# Autodesk Inventor assembly: Printer Frame Assembly RevI
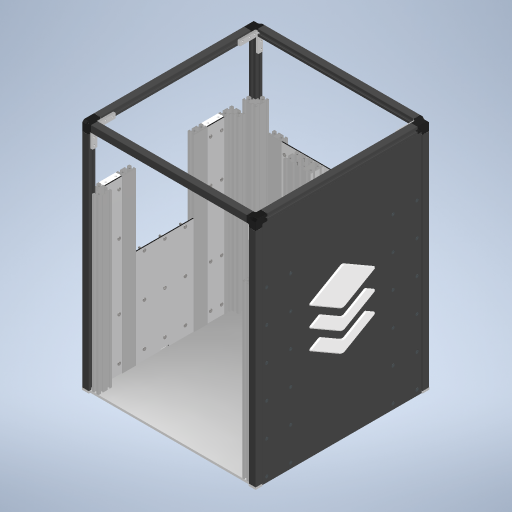
[picture p0: Inventor's stored thumbnail of the model, 512x512]
Saved by Autodesk Inventor 2024 (Build 280153000, 153)
## iProperties
Created: 2024-08-01
Part Number: Printer Frame Assembly RevI
Document SubType Name: Assembly
Designer: Ishaan
Author: Ishaan
## Documents named in this file (16)
- E:\Projects\Axiom--IDEX-3D-Printer\CAD\02 - Frame\Printer Frame Assembly RevI.iam
- E:\Projects\Axiom--IDEX-3D-Printer\CAD\02 - Frame\Printer Base Plate RevI.ipt
- E:\Projects\Axiom--IDEX-3D-Printer\CAD\00 - COTS Components\4040 Vertical L Extrusions\HFS5-404020-500.ipt
- E:\Projects\Axiom--IDEX-3D-Printer\CAD\00 - COTS Components\2040 Vertical Extrusions\HFSF5-2040-500.ipt
- E:\Projects\Axiom--IDEX-3D-Printer\CAD\00 - COTS Components\4080 Z-rail Extrusion\HFSP5-4080-500.ipt
- E:\Projects\Axiom--IDEX-3D-Printer\CAD\00 - COTS Components\2020 Frame Exterior Corners\HFSTB5-2020-650.ipt
- E:\Projects\Axiom--IDEX-3D-Printer\CAD\02 - Frame\Top Corner Extrusion Plate.ipt
- E:\Projects\Axiom--IDEX-3D-Printer\CAD\00 - COTS Components\2020 Frame Exterior X Runners\HFSTB5-2020-456.ipt
- E:\Projects\Axiom--IDEX-3D-Printer\CAD\00 - COTS Components\2020 Frame Exterior Y Runners\HFSFB5-2020-440.ipt
- E:\Projects\Axiom--IDEX-3D-Printer\CAD\02 - Frame\Exterior Frame Corner.ipt
- E:\Projects\Axiom--IDEX-3D-Printer\CAD\02 - Frame\Exterior Frame Corner Other.ipt
- E:\Projects\Axiom--IDEX-3D-Printer\CAD\08 - Side Panelling\Internal Narrow Panels.iam
- E:\Projects\Axiom--IDEX-3D-Printer\CAD\08 - Side Panelling\Internal Wide Panels.iam
- E:\Projects\Axiom--IDEX-3D-Printer\CAD\08 - Side Panelling\Internal Rear Panels.iam
- E:\Projects\Axiom--IDEX-3D-Printer\CAD\08 - Side Panelling\Exterior Side Panels.ipt
- E:\Projects\Axiom--IDEX-3D-Printer\CAD\00 - COTS Components\Hardware\FSCM5x8.ipt
## Components (62 placed, 15 different names)
1. Printer Base Plate RevI:1 — Insert:29, Flush:1, Insert:30, Flush:2, Insert:31, Flush:3, Insert:32, Flush:4, Insert:41, Insert:42, Insert:43, Insert:44, Insert:45, Insert:46, Insert:47, Insert:48, Insert:49, Insert:50, Insert:51, Insert:52, Insert:53, Insert:54, Insert:55, Insert:56, Insert:57, Insert:58, Mate:32
2. HFSF5-2040-500:1
3. HFSF5-2040-500:2 — Mate:33
4. HFSF5-2040-500:3 — Mate:30
5. HFSF5-2040-500:4 — Mate:31
6. HFS5-404020-500:1
7. HFS5-404020-500:2
8. HFS5-404020-500:3
9. HFS5-404020-500:4
10. HFS5-404020-500:5
11. HFS5-404020-500:6
12. HFSP5-4080-500:1 — Mate:29
13. HFSTB5-2020-650:1 — Mate:1, Flush:14, Insert:30, Flush:2, Mate:13
14. HFSTB5-2020-650:2 — Mate:3, Mate:11, Mate:12, Insert:29, Flush:1, Mate:34
15. HFSTB5-2020-650:3 — Mate:2, Flush:15, Insert:32, Flush:4, Mate:14
16. HFSTB5-2020-650:4 — Mate:4, Mate:5, Mate:6, Insert:31, Flush:3
17. Top Corner Extrusion Plate:1 — Mate:1, Flush:14, Mate:13, Insert:34, Angle:1, Mate:18, Insert:39, Mate:21
18. Top Corner Extrusion Plate:2 — Mate:2, Flush:15, Mate:14, Insert:35, Mate:16, Insert:40, Mate:22
19. Top Corner Extrusion Plate:3 — Mate:3, Mate:11, Mate:12, Insert:36, Angle:2, Mate:15, Insert:37, Mate:19
20. Top Corner Extrusion Plate:4 — Mate:4, Mate:5, Mate:6, Insert:33, Mate:17, Insert:38, Mate:20
21. HFSTB5-2020-456:1 — Insert:33, Insert:34, Angle:1
22. HFSTB5-2020-456:2 — Insert:35, Insert:36, Angle:2, Flush:16, Flush:17
23. HFSFB5-2020-440:1 — Mate:15, Flush:16, Mate:18, Mate:35
24. HFSFB5-2020-440:2 — Flush:17, Mate:16, Mate:17
25. Exterior Frame Corner:1 — Insert:37, Mate:19
26. Exterior Frame Corner:2 — Insert:38, Mate:20
27. Exterior Frame Corner Other:1 — Insert:39, Mate:21
28. Exterior Frame Corner Other:2 — Insert:40, Mate:22
29. HFSF5-2040-500:5 — Insert:43, Insert:44
30. HFSF5-2040-500:6 — Insert:41, Insert:42
31. Internal Narrow Panels:1 [sub-assembly] — Insert:51, Insert:52
32. Internal Narrow Panels:2 [sub-assembly] — Insert:49, Insert:50
33. Internal Narrow Panels:3 [sub-assembly] — Insert:47, Insert:48
34. Internal Narrow Panels:4 [sub-assembly] — Insert:45, Insert:46
35. Internal Wide Panels:1 [sub-assembly] — Insert:53, Insert:54, Insert:55
36. Internal Wide Panels:2 [sub-assembly] — Insert:56, Insert:57, Insert:58
37. Internal Rear Panels:1 [sub-assembly] — Mate:29, Mate:30, Mate:31, Mate:32
38. Exterior Side Panels:1 — Mate:33, Mate:34, Mate:35, Insert:59, Insert:60, Insert:61, Insert:62, Insert:63, Insert:64, Insert:65, Insert:66, Insert:67, Insert:68, Insert:69, Insert:70, Insert:71, Insert:72, Insert:73, Insert:74, Insert:75, Insert:76, Insert:77, Insert:78, Insert:79, Insert:80, Insert:81, Insert:82
39. FSCM5x8:1 — Insert:64
40. FSCM5x8:2 — Insert:63
41. FSCM5x8:3 — Insert:62
42. FSCM5x8:4 — Insert:61
43. FSCM5x8:5 — Insert:60
44. FSCM5x8:6 — Insert:59
45. FSCM5x8:7 — Insert:65
46. FSCM5x8:8 — Insert:66
47. FSCM5x8:9 — Insert:67
48. FSCM5x8:10 — Insert:68
49. FSCM5x8:11 — Insert:69
50. FSCM5x8:12 — Insert:70
51. FSCM5x8:13 — Insert:76
52. FSCM5x8:14 — Insert:75
53. FSCM5x8:15 — Insert:74
54. FSCM5x8:16 — Insert:73
55. FSCM5x8:17 — Insert:72
56. FSCM5x8:18 — Insert:71
57. FSCM5x8:19 — Insert:77
58. FSCM5x8:20 — Insert:78
59. FSCM5x8:21 — Insert:79
60. FSCM5x8:22 — Insert:80
61. FSCM5x8:23 — Insert:81
62. FSCM5x8:24 — Insert:82
## Relationships (117: Insert 82, Mate 25, Flush 8, Angle 2)
- [Insert]: Printer Base Plate RevI:1 ↔ HFSF5-2040-500:4
- [Insert]: Printer Base Plate RevI:1 ↔ HFSF5-2040-500:4
- [Insert]: Printer Base Plate RevI:1 ↔ HFSF5-2040-500:3
- [Insert]: Printer Base Plate RevI:1 ↔ HFSF5-2040-500:3
- [Insert]: Printer Base Plate RevI:1 ↔ HFSF5-2040-500:2
- [Insert]: Printer Base Plate RevI:1 ↔ HFSF5-2040-500:2
- [Insert]: Printer Base Plate RevI:1 ↔ HFSF5-2040-500:1
- [Insert]: Printer Base Plate RevI:1 ↔ HFSF5-2040-500:1
- [Insert]: Printer Base Plate RevI:1 ↔ HFS5-404020-500:6
- [Insert]: Printer Base Plate RevI:1 ↔ HFS5-404020-500:6
- [Insert]: Printer Base Plate RevI:1 ↔ HFS5-404020-500:5
- [Insert]: Printer Base Plate RevI:1 ↔ HFS5-404020-500:5
- [Insert]: Printer Base Plate RevI:1 ↔ HFS5-404020-500:4
- [Insert]: Printer Base Plate RevI:1 ↔ HFS5-404020-500:4
- [Insert]: Printer Base Plate RevI:1 ↔ HFS5-404020-500:3
- [Insert]: Printer Base Plate RevI:1 ↔ HFS5-404020-500:3
- [Insert]: Printer Base Plate RevI:1 ↔ HFS5-404020-500:2
- [Insert]: Printer Base Plate RevI:1 ↔ HFS5-404020-500:2
- [Insert]: Printer Base Plate RevI:1 ↔ HFS5-404020-500:1
- [Insert]: Printer Base Plate RevI:1 ↔ HFS5-404020-500:1
- [Insert]: Printer Base Plate RevI:1 ↔ HFSP5-4080-500:1
- [Insert]: Printer Base Plate RevI:1 ↔ HFSP5-4080-500:1
- [Insert]: Printer Base Plate RevI:1 ↔ HFSP5-4080-500:1
- [Insert]: Printer Base Plate RevI:1 ↔ HFSP5-4080-500:1
- [Insert]: Printer Base Plate RevI:1 ↔ HFSP5-4080-500:1
- [Insert]: Printer Base Plate RevI:1 ↔ HFSP5-4080-500:1
- [Insert]: Printer Base Plate RevI:1 ↔ HFSP5-4080-500:1
- [Insert]: Printer Base Plate RevI:1 ↔ HFSP5-4080-500:1
- Mate:1: HFSTB5-2020-650:1 ↔ Top Corner Extrusion Plate:1
- Mate:2: HFSTB5-2020-650:3 ↔ Top Corner Extrusion Plate:2
- Mate:3: HFSTB5-2020-650:2 ↔ Top Corner Extrusion Plate:3
- Mate:4: HFSTB5-2020-650:4 ↔ Top Corner Extrusion Plate:4
- Mate:5: HFSTB5-2020-650:4 ↔ Top Corner Extrusion Plate:4
- Mate:6 (9 mm): HFSTB5-2020-650:4 ↔ Top Corner Extrusion Plate:4
- Flush:14: HFSTB5-2020-650:1 ↔ Top Corner Extrusion Plate:1
- Flush:15: HFSTB5-2020-650:3 ↔ Top Corner Extrusion Plate:2
- Mate:11: HFSTB5-2020-650:2 ↔ Top Corner Extrusion Plate:3
- Mate:12 (9 mm): HFSTB5-2020-650:2 ↔ Top Corner Extrusion Plate:3
- Insert:29: Printer Base Plate RevI:1 ↔ HFSTB5-2020-650:2
- Flush:1: Printer Base Plate RevI:1 ↔ HFSTB5-2020-650:2
- Insert:30: Printer Base Plate RevI:1 ↔ HFSTB5-2020-650:1
- Flush:2: Printer Base Plate RevI:1 ↔ HFSTB5-2020-650:1
- Insert:31: Printer Base Plate RevI:1 ↔ HFSTB5-2020-650:4
- Flush:3: Printer Base Plate RevI:1 ↔ HFSTB5-2020-650:4
- Insert:32: Printer Base Plate RevI:1 ↔ HFSTB5-2020-650:3
- Flush:4: Printer Base Plate RevI:1 ↔ HFSTB5-2020-650:3
- Mate:13 (9 mm): HFSTB5-2020-650:1 ↔ Top Corner Extrusion Plate:1
- Mate:14 (9 mm): HFSTB5-2020-650:3 ↔ Top Corner Extrusion Plate:2
- Insert:33: Top Corner Extrusion Plate:4 ↔ HFSTB5-2020-456:1
- Insert:34: Top Corner Extrusion Plate:1 ↔ HFSTB5-2020-456:1
- Angle:1 (0 deg): Top Corner Extrusion Plate:1 ↔ HFSTB5-2020-456:1
- Insert:35: Top Corner Extrusion Plate:2 ↔ HFSTB5-2020-456:2
- Insert:36: Top Corner Extrusion Plate:3 ↔ HFSTB5-2020-456:2
- Angle:2 (0 deg): Top Corner Extrusion Plate:3 ↔ HFSTB5-2020-456:2
- Mate:15: Top Corner Extrusion Plate:3 ↔ HFSFB5-2020-440:1
- Flush:16: HFSTB5-2020-456:2 ↔ HFSFB5-2020-440:1
- Flush:17: HFSTB5-2020-456:2 ↔ HFSFB5-2020-440:2
- Mate:16: Top Corner Extrusion Plate:2 ↔ HFSFB5-2020-440:2
- Mate:17 (-38 mm): Top Corner Extrusion Plate:4 ↔ HFSFB5-2020-440:2
- Mate:18 (-38 mm): Top Corner Extrusion Plate:1 ↔ HFSFB5-2020-440:1
- Insert:37: Top Corner Extrusion Plate:3 ↔ Exterior Frame Corner:1
- Mate:19: Top Corner Extrusion Plate:3 ↔ Exterior Frame Corner:1
- Insert:38: Top Corner Extrusion Plate:4 ↔ Exterior Frame Corner:2
- Mate:20: Top Corner Extrusion Plate:4 ↔ Exterior Frame Corner:2
- Insert:39: Top Corner Extrusion Plate:1 ↔ Exterior Frame Corner Other:1
- Mate:21: Top Corner Extrusion Plate:1 ↔ Exterior Frame Corner Other:1
- Insert:40: Top Corner Extrusion Plate:2 ↔ Exterior Frame Corner Other:2
- Mate:22: Top Corner Extrusion Plate:2 ↔ Exterior Frame Corner Other:2
- Insert:41: Printer Base Plate RevI:1 ↔ HFSF5-2040-500:6
- Insert:42: Printer Base Plate RevI:1 ↔ HFSF5-2040-500:6
- Insert:43: Printer Base Plate RevI:1 ↔ HFSF5-2040-500:5
- Insert:44: Printer Base Plate RevI:1 ↔ HFSF5-2040-500:5
- Insert:45: Printer Base Plate RevI:1 ↔ Internal Narrow Panels:4
- Insert:46: Printer Base Plate RevI:1 ↔ Internal Narrow Panels:4
- Insert:47: Printer Base Plate RevI:1 ↔ Internal Narrow Panels:3
- Insert:48: Printer Base Plate RevI:1 ↔ Internal Narrow Panels:3
- Insert:49: Printer Base Plate RevI:1 ↔ Internal Narrow Panels:2
- Insert:50: Printer Base Plate RevI:1 ↔ Internal Narrow Panels:2
- Insert:51: Printer Base Plate RevI:1 ↔ Internal Narrow Panels:1
- Insert:52: Printer Base Plate RevI:1 ↔ Internal Narrow Panels:1
- Insert:53: Printer Base Plate RevI:1 ↔ Internal Wide Panels:1
- Insert:54: Printer Base Plate RevI:1 ↔ Internal Wide Panels:1
- Insert:55: Printer Base Plate RevI:1 ↔ Internal Wide Panels:1
- Insert:56: Printer Base Plate RevI:1 ↔ Internal Wide Panels:2
- Insert:57: Printer Base Plate RevI:1 ↔ Internal Wide Panels:2
- Insert:58: Printer Base Plate RevI:1 ↔ Internal Wide Panels:2
- Mate:29: HFSP5-4080-500:1 ↔ Internal Rear Panels:1
- Mate:30: HFSF5-2040-500:3 ↔ Internal Rear Panels:1
- Mate:31: HFSF5-2040-500:4 ↔ Internal Rear Panels:1
- Mate:32 (0.5 mm): Printer Base Plate RevI:1 ↔ Internal Rear Panels:1
- Mate:33: HFSF5-2040-500:2 ↔ Exterior Side Panels:1
- Mate:34 (1 mm): HFSTB5-2020-650:2 ↔ Exterior Side Panels:1
- Mate:35 (1 mm): HFSFB5-2020-440:1 ↔ Exterior Side Panels:1
- Insert:59: Exterior Side Panels:1 ↔ FSCM5x8:6
- Insert:60: Exterior Side Panels:1 ↔ FSCM5x8:5
- Insert:61: Exterior Side Panels:1 ↔ FSCM5x8:4
- Insert:62: Exterior Side Panels:1 ↔ FSCM5x8:3
- Insert:63: Exterior Side Panels:1 ↔ FSCM5x8:2
- Insert:64: Exterior Side Panels:1 ↔ FSCM5x8:1
- Insert:65: Exterior Side Panels:1 ↔ FSCM5x8:7
- Insert:66: Exterior Side Panels:1 ↔ FSCM5x8:8
- Insert:67: Exterior Side Panels:1 ↔ FSCM5x8:9
- Insert:68: Exterior Side Panels:1 ↔ FSCM5x8:10
- Insert:69: Exterior Side Panels:1 ↔ FSCM5x8:11
- Insert:70: Exterior Side Panels:1 ↔ FSCM5x8:12
- Insert:71: Exterior Side Panels:1 ↔ FSCM5x8:18
- Insert:72: Exterior Side Panels:1 ↔ FSCM5x8:17
- Insert:73: Exterior Side Panels:1 ↔ FSCM5x8:16
- Insert:74: Exterior Side Panels:1 ↔ FSCM5x8:15
- Insert:75: Exterior Side Panels:1 ↔ FSCM5x8:14
- Insert:76: Exterior Side Panels:1 ↔ FSCM5x8:13
- Insert:77: Exterior Side Panels:1 ↔ FSCM5x8:19
- Insert:78: Exterior Side Panels:1 ↔ FSCM5x8:20
- Insert:79: Exterior Side Panels:1 ↔ FSCM5x8:21
- Insert:80: Exterior Side Panels:1 ↔ FSCM5x8:22
- Insert:81: Exterior Side Panels:1 ↔ FSCM5x8:23
- Insert:82: Exterior Side Panels:1 ↔ FSCM5x8:24
